# Autodesk Inventor assembly: TheClaw
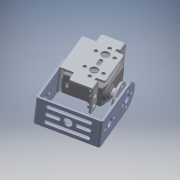
[picture p0: Inventor's stored thumbnail of the model, 180x180]
Saved by Autodesk Inventor 2017 (Build 210142000, 142)
## iProperties
Created: 2017-09-30
Part Number: TheClaw
Document SubType Name: Assembly
Designer: User
Author: User
## Documents named in this file (5)
- C:\Robotics\CAD\2017-18_CAD\Miscellaneous\TheClaw.iam
- C:\Robotics\CAD\COTSParts\Tetrix\39593_txm-standard-scale pivot armwbearing..ipt
- C:\Robotics\CAD\COTSParts\Tetrix\39020_txm-servo mount horn.ipt
- C:\Robotics\CAD\COTSParts\Rev\REV-41-1097.ipt
- C:\Robotics\CAD\COTSParts\Tetrix\39060_txm-standard servo bracket.ipt
## Components (4 placed, 4 different names)
1. 39593_txm-standard-scale pivot armwbearing.:1 — Mate:37, Mate:42, Mate:45, Angle:2
2. 39020_txm-servo mount horn:1 — Mate:23, Mate:24
3. REV-41-1097:2 — Mate:23, Mate:24, Insert:3, Insert:4
4. 39060_txm-standard servo bracket:1 — Mate:37, Mate:42, Mate:45, Insert:3, Insert:4, Angle:2
## Relationships (8: Mate 5, Insert 2, Angle 1)
- Mate:23: 39020_txm-servo mount horn:1 ↔ REV-41-1097:2
- Mate:24: 39020_txm-servo mount horn:1 ↔ REV-41-1097:2
- Mate:37: 39593_txm-standard-scale pivot armwbearing.:1 ↔ 39060_txm-standard servo bracket:1
- Mate:42: 39593_txm-standard-scale pivot armwbearing.:1 ↔ 39060_txm-standard servo bracket:1
- Mate:45: 39593_txm-standard-scale pivot armwbearing.:1 ↔ 39060_txm-standard servo bracket:1
- Insert:3: REV-41-1097:2 ↔ 39060_txm-standard servo bracket:1
- Insert:4: REV-41-1097:2 ↔ 39060_txm-standard servo bracket:1
- Angle:2 (0 deg): 39593_txm-standard-scale pivot armwbearing.:1 ↔ 39060_txm-standard servo bracket:1
